# Autodesk Inventor assembly: Tower Assm
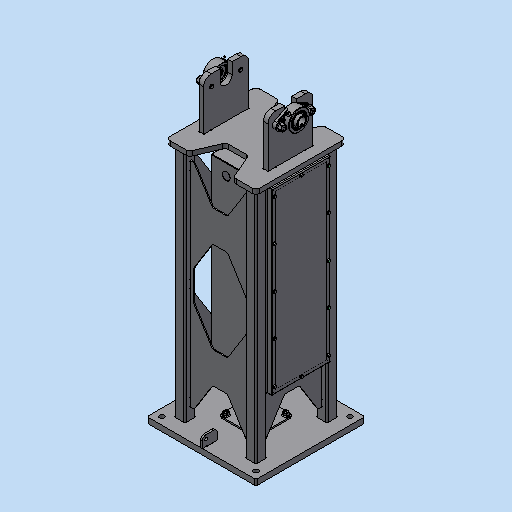
[picture p0: Inventor's stored thumbnail of the model, 512x512]
Saved by Autodesk Inventor 2025.3 (Build 293356030, 356C)
## iProperties
RuleStatus: InUse
Created: 2025-09-18
Part Number: Tower Assm
Document SubType Name: Assembly
Designer: titus
Description: Cleaning Robot Tower Assembly
Mass: 62310.8 g
Surface Area: 35204 cm^2
Volume: 7937.69 cm^3
Density: 7.85 g/cm^3
Author: titus
## Documents named in this file (10)
- R:\A1- Neuweg Design Data\OM Robotics\CLEANING ROBOT TOWER PROJECT\Tower Assm.iam
- R:\A1- Neuweg Design Data\OM Robotics\CLEANING ROBOT TOWER PROJECT\ELB-ASM-1001.iam
- R:\A1- Neuweg Design Data\OM Robotics\CLEANING ROBOT TOWER PROJECT\92979A340.ipt
- R:\A1- Neuweg Design Data\OM Robotics\CLEANING ROBOT TOWER PROJECT\ELB-ASM-1000.iam
- R:\A1- Neuweg Design Data\OM Robotics\CLEANING ROBOT TOWER PROJECT\5968K75.ipt
- R:\A1- Neuweg Design Data\OM Robotics\CLEANING ROBOT TOWER PROJECT\92979A114.ipt
- R:\A1- Neuweg Design Data\OM Robotics\CLEANING ROBOT TOWER PROJECT\ELB-ASM-1002.iam
- R:\A1- Neuweg Design Data\OM Robotics\CLEANING ROBOT TOWER PROJECT\92979A467.ipt
- R:\A1- Neuweg Design Data\OM Robotics\CLEANING ROBOT TOWER PROJECT\95615A120.ipt
- R:\A1- Neuweg Design Data\OM Robotics\CLEANING ROBOT TOWER PROJECT\90096A334.ipt
## Components (27 placed, 9 different names)
1. ELB-ASM-1002:1 [sub-assembly] — Mate:1, Mate:2, Mate:3, Mate:4, Mate:5, Mate:6, Mate:7, Mate:8, Mate:9, Mate:10, Mate:11
2. ELB-ASM-1001:1 [sub-assembly] — Insert:3, Insert:4, Insert:5, Insert:6, Insert:7, Insert:8, Mate:1, Mate:2, Insert:23, Insert:24, Insert:25, Insert:26
3. 92979A340:1 — Insert:3
4. 92979A340:2 — Insert:4
5. 92979A340:3 — Insert:5, Mate:3
6. 92979A340:4 — Insert:6
7. ELB-ASM-1000:1 [sub-assembly] — Insert:7, Insert:8, Insert:19, Insert:20, Insert:21, Insert:22, Insert:27, Insert:28, Insert:29, Insert:30, Insert:31, Insert:32
8. 5968K75:1 — Mate:8, Mate:9, Mate:10, Mate:11, Insert:15, Insert:16
9. 5968K75:2 — Mate:4, Mate:5, Mate:6, Mate:7, Insert:17, Insert:18
10. 92979A467:1 — Insert:15
11. 92979A467:2 — Insert:17
12. 92979A467:3 — Insert:18
13. 92979A467:4 — Insert:16
14. 92979A114:7 — Insert:19
15. 92979A114:8 — Insert:22
16. 92979A114:9 — Insert:20
17. 92979A114:10 — Insert:21
18. 95615A120:1 — Insert:24
19. 95615A120:2 — Insert:23
20. 95615A120:3 — Insert:26
21. 95615A120:4 — Insert:25
22. 90096A334:1 — Insert:27
23. 90096A334:2 — Insert:28
24. 90096A334:3 — Insert:29
25. 90096A334:4 — Insert:30
26. 90096A334:5 — Insert:32
27. 90096A334:6 — Insert:31
## Relationships (35: Insert 24, Mate 11)
- Insert:3: ELB-ASM-1001:1 ↔ 92979A340:1
- Insert:4: ELB-ASM-1001:1 ↔ 92979A340:2
- Insert:5: ELB-ASM-1001:1 ↔ 92979A340:3
- Insert:6: ELB-ASM-1001:1 ↔ 92979A340:4
- Insert:7: ELB-ASM-1001:1 ↔ ELB-ASM-1000:1
- Insert:8: ELB-ASM-1001:1 ↔ ELB-ASM-1000:1
- Mate:1: ELB-ASM-1002:1 ↔ ELB-ASM-1001:1
- Mate:2: ELB-ASM-1002:1 ↔ ELB-ASM-1001:1
- Mate:3: ELB-ASM-1002:1 ↔ 92979A340:3
- Mate:4: ELB-ASM-1002:1 ↔ 5968K75:2
- Mate:5: ELB-ASM-1002:1 ↔ 5968K75:2
- Mate:6: ELB-ASM-1002:1 ↔ 5968K75:2
- Mate:7: ELB-ASM-1002:1 ↔ 5968K75:2
- Mate:8: ELB-ASM-1002:1 ↔ 5968K75:1
- Mate:9: ELB-ASM-1002:1 ↔ 5968K75:1
- Mate:10: ELB-ASM-1002:1 ↔ 5968K75:1
- Mate:11: ELB-ASM-1002:1 ↔ 5968K75:1
- Insert:15: 5968K75:1 ↔ 92979A467:1
- Insert:16: 5968K75:1 ↔ 92979A467:4
- Insert:17: 5968K75:2 ↔ 92979A467:2
- Insert:18: 5968K75:2 ↔ 92979A467:3
- Insert:19: ELB-ASM-1000:1 ↔ 92979A114:7
- Insert:20: ELB-ASM-1000:1 ↔ 92979A114:9
- Insert:21: ELB-ASM-1000:1 ↔ 92979A114:10
- Insert:22: ELB-ASM-1000:1 ↔ 92979A114:8
- Insert:23: ELB-ASM-1001:1 ↔ 95615A120:2
- Insert:24: ELB-ASM-1001:1 ↔ 95615A120:1
- Insert:25: ELB-ASM-1001:1 ↔ 95615A120:4
- Insert:26: ELB-ASM-1001:1 ↔ 95615A120:3
- Insert:27: ELB-ASM-1000:1 ↔ 90096A334:1
- Insert:28: ELB-ASM-1000:1 ↔ 90096A334:2
- Insert:29: ELB-ASM-1000:1 ↔ 90096A334:3
- Insert:30: ELB-ASM-1000:1 ↔ 90096A334:4
- Insert:31: ELB-ASM-1000:1 ↔ 90096A334:6
- Insert:32: ELB-ASM-1000:1 ↔ 90096A334:5
